# Autodesk Inventor assembly: VNA-Port2-Kabelfixierung
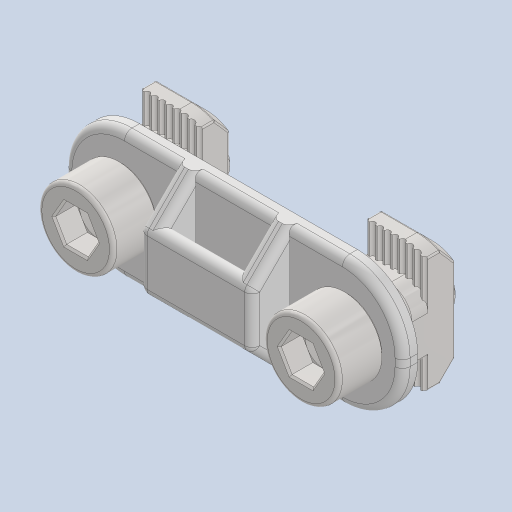
[picture p0: Inventor's stored thumbnail of the model, 512x512]
Saved by Autodesk Inventor 2023.2 (Build 272271000, 271)
## iProperties
Created: 2024-07-03
Part Number: VNA-Port2-Kabelfixierung
Document SubType Name: Assembly
Designer: Nils Bade
Author: Nils Bade
## Documents named in this file (4)
- C:\Users\nilsb\Documents\Inventor\Projektarbeit-Bade\RatRig_modified\VNA-Port2-Kabelfixierung.iam
- C:\Users\nilsb\Documents\Inventor\Projektarbeit-Bade\RatRig_modified\VNA-Port2-Kabelfixierung.ipt
- C:\Users\nilsb\Documents\Inventor\Projektarbeit-Bade\Schrauben\Cap Head Screw M6x12 v2.ipt
- C:\Users\nilsb\Documents\Inventor\Projektarbeit-Bade\RatRig_Standards\T-Nut - Drop In for 3030 - M6 v2.ipt
## Components (5 placed, 3 different names)
1. VNA-Port2-Kabelfixierung:1 — Passend:1, Passend:2, Passend:3, Passend:4, Winkel:1, Winkel:2, Passend:7, Passend:8
2. Cap Head Screw M6x12 v2:1 — Passend:1, Passend:3, Passend:6
3. Cap Head Screw M6x12 v2:2 — Passend:2, Passend:4, Passend:5
4. T-Nut - Drop In for 3030 - M6 v2:1 — Passend:5, Winkel:2, Passend:7
5. T-Nut - Drop In for 3030 - M6 v2:2 — Passend:6, Winkel:1, Passend:8
## Relationships (10: Mate 8, Angle 2)
- Passend:1 [Mate]: VNA-Port2-Kabelfixierung:1 ↔ Cap Head Screw M6x12 v2:1
- Passend:2 [Mate]: VNA-Port2-Kabelfixierung:1 ↔ Cap Head Screw M6x12 v2:2
- Passend:3 [Mate]: VNA-Port2-Kabelfixierung:1 ↔ Cap Head Screw M6x12 v2:1
- Passend:4 [Mate]: VNA-Port2-Kabelfixierung:1 ↔ Cap Head Screw M6x12 v2:2
- Passend:5 [Mate]: Cap Head Screw M6x12 v2:2 ↔ T-Nut - Drop In for 3030 - M6 v2:1
- Passend:6 [Mate]: Cap Head Screw M6x12 v2:1 ↔ T-Nut - Drop In for 3030 - M6 v2:2
- Winkel:1 [Angle] (0 deg): VNA-Port2-Kabelfixierung:1 ↔ T-Nut - Drop In for 3030 - M6 v2:2
- Winkel:2 [Angle] (0 deg): VNA-Port2-Kabelfixierung:1 ↔ T-Nut - Drop In for 3030 - M6 v2:1
- Passend:7 [Mate] (4.5 mm): VNA-Port2-Kabelfixierung:1 ↔ T-Nut - Drop In for 3030 - M6 v2:1
- Passend:8 [Mate] (4.5 mm): VNA-Port2-Kabelfixierung:1 ↔ T-Nut - Drop In for 3030 - M6 v2:2
